# Autodesk Inventor assembly: ENSAMBLAJE_VENTOSA_1
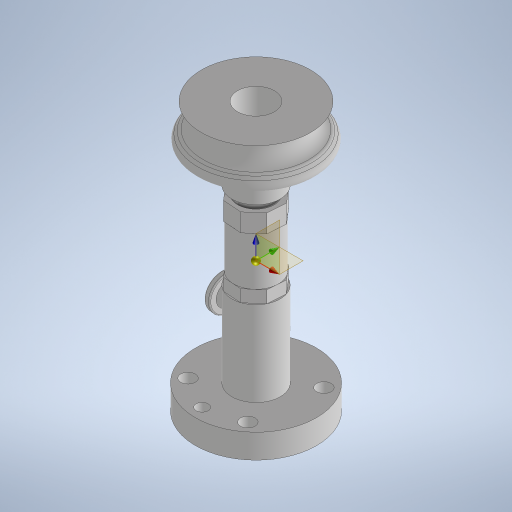
[picture p0: Inventor's stored thumbnail of the model, 512x512]
Saved by Autodesk Inventor 2024 (Build 280153000, 153)
## iProperties
Created: 2022-10-31
Part Number: ENSAMBLAJE_VENTOSA_1
Document SubType Name: Assembly
Designer: Usuario
Mass: 57.9805 g
Surface Area: 254.277 cm^2
Volume: 57.9805 cm^3
Density: 1 g/cm^3
Author: Usuario
## Documents named in this file (5)
- C:\Users\sebas\OneDrive\Documentos\Cosas de Sebastian\APM\Esdek\Celda Robotizada\ROBOT STUDIO\CAD\HERRAMIENTA\ENSAMBLAJE_VENTOSA_1.iam
- C:\Users\sebas\OneDrive\Documentos\Cosas de Sebastian\APM\Esdek\Celda Robotizada\ROBOT STUDIO\CAD\HERRAMIENTA\TORNILLO.ipt
- C:\Users\sebas\OneDrive\Documentos\Cosas de Sebastian\APM\Esdek\Celda Robotizada\ROBOT STUDIO\CAD\HERRAMIENTA\TUBO_METALICO.ipt
- C:\Users\sebas\OneDrive\Documentos\Cosas de Sebastian\APM\Esdek\Celda Robotizada\ROBOT STUDIO\CAD\HERRAMIENTA\VENTOSA.ipt
- C:\Users\sebas\OneDrive\Documentos\Cosas de Sebastian\APM\Esdek\Celda Robotizada\ROBOT STUDIO\CAD\HERRAMIENTA\ACOPLE.ipt
## Components (4 placed, 4 different names)
1. TORNILLO:1 — Cilíndrica:1
2. TUBO_METALICO:1 — Coincidencia:2
3. VENTOSA:1 — Coincidencia:4
4. ACOPLE:1 — Cilíndrica:1, Coincidencia:2, Coincidencia:3
## Relationships (7: Mate 4, RevoluteJoint 1, Insert 1, CylindricalJoint 1)
- [RevoluteJoint]: TORNILLO:1 ↔ VENTOSA:1
- [Insert] (-21 mm): TORNILLO:1 ↔ TUBO_METALICO:1
- [Mate]: TORNILLO:1 ↔ VENTOSA:1
- Cilíndrica:1 [CylindricalJoint]: TORNILLO:1 ↔ ACOPLE:1
- Coincidencia:2 [Mate]: TUBO_METALICO:1 ↔ ACOPLE:1
- Coincidencia:3 [Mate]: ACOPLE:1
- Coincidencia:4 [Mate]: VENTOSA:1
